# Autodesk Inventor assembly: chassis
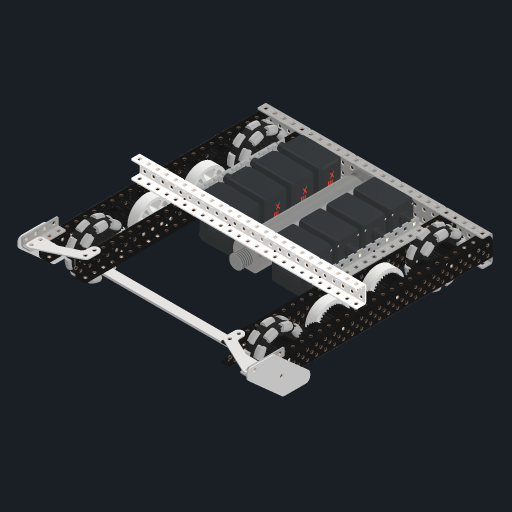
[picture p0: Inventor's stored thumbnail of the model, 512x512]
Saved by Autodesk Inventor 2024.2 (Build 282272000, 272)
## iProperties
Created: 2024-01-28
Part Number: chassis
Document SubType Name: Assembly
Designer: reima
Mass: 1228.84 g
Surface Area: 6404.9 cm^2
Volume: 505.466 cm^3
Density: 2.43111 g/cm^3
Author: reima
## Documents named in this file (15)
- O:\cad\61002g-cad\subasm\chassis.iam
- O:\cad\61002g-cad\VEX parts\Structure\C Channel\Aluminum 1x2x1\Alu C 1x2x1x25.ipt
- O:\cad\61002g-cad\VEX parts\Structure\C Channel\Aluminum 1x3x1\Alu C 1x3x1x25.ipt
- O:\cad\61002g-cad\subasm\omniAsemb.iam
- O:\cad\61002g-cad\subasm\flexMid.iam
- O:\cad\61002g-cad\VEX parts\Motion\Gears\LS 36T Gear.ipt
- O:\cad\61002g-cad\plastic parts\6inSleds.ipt
- O:\cad\61002g-cad\VEX parts\Structure\Angle\Aluminum 1x1\Alu Angle 1x1x4.ipt
- O:\cad\61002g-cad\plastic parts\frontgussets.ipt
- O:\cad\61002g-cad\VEX parts\Electronics\V5 Motor.ipt
- O:\cad\61002g-cad\plastic parts\undersideStrip.ipt
- O:\cad\61002g-cad\VEX parts\Structure\C Channel\Aluminum 1x2x1 Half\Alu Half C 1x2x1x10\Alu Half C 1x2x1x10.ipt
- O:\cad\61002g-cad\VEX parts\Structure\C Channel\Aluminum 1x2x1 Half\Alu Half C 1x2x1x10.ipt
- O:\cad\61002g-cad\VEX parts\Motion\Pneumatics\Reservoir.ipt
- O:\cad\61002g-cad\VEX parts\Miscellaneous\iw_metal_02.bmp
## Components (38 placed, 12 different names)
1. Alu C 1x2x1x25:1 — Insert:2, Mate:2, Insert:14, Insert:15, Insert:16, Insert:17, Mate:7, Mate:10, Flush:6, Flush:7, Insert:35
2. Alu C 1x2x1x25:2 — Insert:1, Mate:2, Insert:5, Insert:6, Insert:7, Insert:8, Insert:9, Insert:10, Insert:11, Insert:12, Angle:1, Insert:13, Mate:3, Mate:8
3. Alu C 1x3x1x25:1 — Insert:1, Insert:2, Angle:2, Flush:3, Insert:31
4. omniAsemb:3 [sub-assembly] — Insert:5
5. omniAsemb:6 [sub-assembly] — Insert:11
6. LS 36T Gear:4 — Insert:6
7. flexMid:5 [sub-assembly] — Insert:7
8. flexMid:6 [sub-assembly] — Insert:9
9. LS 36T Gear:5 — Insert:8
10. LS 36T Gear:6 — Insert:10
11. 6inSleds:2 — Insert:12, Angle:1
12. Alu Angle 1x1x4:1 — Insert:13, Mate:3
13. frontgussets:2 — Insert:14
14. V5 Motor:1 — Insert:15
15. V5 Motor:2 — Insert:16
16. V5 Motor:3 — Insert:17
17. Alu C 1x2x1x25:3 — Mate:5, Insert:27, Insert:28, Insert:29, Insert:30, Insert:33, Mate:9, Flush:4, Flush:5, Insert:36
18. Alu C 1x2x1x25:4 — Mate:5, Insert:18, Insert:19, Insert:20, Insert:21, Insert:22, Insert:23, Insert:24, Insert:25, Angle:3, Mate:6, Insert:26, Insert:31, Insert:34
19. omniAsemb:7 [sub-assembly] — Insert:18
20. omniAsemb:8 [sub-assembly] — Insert:19
21. LS 36T Gear:7 — Insert:20
22. flexMid:7 [sub-assembly] — Insert:21
23. flexMid:8 [sub-assembly] — Insert:22
24. LS 36T Gear:8 — Insert:23
25. LS 36T Gear:9 — Insert:24
26. 6inSleds:3 — Insert:25, Angle:3
27. Alu Angle 1x1x4:2 — Mate:6, Insert:26, Insert:32
28. frontgussets:3 — Insert:27, Insert:32
29. V5 Motor:4 — Insert:28
30. V5 Motor:5 — Insert:29
31. V5 Motor:6 — Insert:30
32. undersideStrip:2 — Insert:33, Mate:7
33. Alu C 1x2x1x25:5 — Insert:34, Mate:8, Mate:11, Mate:12
34. Alu Half C 1x2x1x10:1 — Mate:10, Flush:6, Flush:7
35. Alu Half C 1x2x1x10:2 — Mate:9, Flush:4, Flush:5
36. V5 Motor:7 — Insert:35
37. V5 Motor:8 — Insert:36
38. Reservoir:1 — Mate:11, Mate:12
## Relationships (52: Insert 34, Mate 10, Flush 5, Angle 3)
- Insert:1 (3.175 mm): Alu C 1x2x1x25:2 ↔ Alu C 1x3x1x25:1
- Insert:2 (3.175 mm): Alu C 1x2x1x25:1 ↔ Alu C 1x3x1x25:1
- Mate:2: Alu C 1x2x1x25:1 ↔ Alu C 1x2x1x25:2
- Insert:5 (13.4938 mm): Alu C 1x2x1x25:2 ↔ omniAsemb:3
- Insert:6 (13.4938 mm): Alu C 1x2x1x25:2 ↔ LS 36T Gear:4
- Insert:7 (13.4938 mm): Alu C 1x2x1x25:2 ↔ flexMid:5
- Insert:8 (13.4938 mm): Alu C 1x2x1x25:2 ↔ LS 36T Gear:5
- Insert:9 (13.4938 mm): Alu C 1x2x1x25:2 ↔ flexMid:6
- Insert:10 (13.4938 mm): Alu C 1x2x1x25:2 ↔ LS 36T Gear:6
- Insert:11 (13.4938 mm): Alu C 1x2x1x25:2 ↔ omniAsemb:6
- Insert:12: Alu C 1x2x1x25:2 ↔ 6inSleds:2
- Angle:1 (180 deg): Alu C 1x2x1x25:2 ↔ 6inSleds:2
- Insert:13: Alu C 1x2x1x25:2 ↔ Alu Angle 1x1x4:1
- Mate:3: Alu C 1x2x1x25:2 ↔ Alu Angle 1x1x4:1
- Insert:14 (1.5875 mm): Alu C 1x2x1x25:1 ↔ frontgussets:2
- Insert:15 (14.2875 mm): Alu C 1x2x1x25:1 ↔ V5 Motor:1
- Insert:16 (14.2875 mm): Alu C 1x2x1x25:1 ↔ V5 Motor:2
- Insert:17 (14.2875 mm): Alu C 1x2x1x25:1 ↔ V5 Motor:3
- Angle:2 (0 deg): Alu C 1x3x1x25:1
- Flush:3 (158.75 mm): Alu C 1x3x1x25:1
- Mate:5: Alu C 1x2x1x25:3 ↔ Alu C 1x2x1x25:4
- Insert:18 (13.4938 mm): Alu C 1x2x1x25:4 ↔ omniAsemb:7
- Insert:19 (13.4938 mm): Alu C 1x2x1x25:4 ↔ omniAsemb:8
- Insert:20 (13.4938 mm): Alu C 1x2x1x25:4 ↔ LS 36T Gear:7
- Insert:21 (13.4938 mm): Alu C 1x2x1x25:4 ↔ flexMid:7
- Insert:22 (13.4938 mm): Alu C 1x2x1x25:4 ↔ flexMid:8
- Insert:23 (13.4938 mm): Alu C 1x2x1x25:4 ↔ LS 36T Gear:8
- Insert:24 (13.4938 mm): Alu C 1x2x1x25:4 ↔ LS 36T Gear:9
- Insert:25: Alu C 1x2x1x25:4 ↔ 6inSleds:3
- Angle:3 (180 deg): Alu C 1x2x1x25:4 ↔ 6inSleds:3
- Mate:6: Alu C 1x2x1x25:4 ↔ Alu Angle 1x1x4:2
- Insert:26: Alu C 1x2x1x25:4 ↔ Alu Angle 1x1x4:2
- Insert:27 (1.5875 mm): Alu C 1x2x1x25:3 ↔ frontgussets:3
- Insert:28 (14.2875 mm): Alu C 1x2x1x25:3 ↔ V5 Motor:4
- Insert:29 (14.2875 mm): Alu C 1x2x1x25:3 ↔ V5 Motor:5
- Insert:30 (14.2875 mm): Alu C 1x2x1x25:3 ↔ V5 Motor:6
- Insert:31 (3.175 mm): Alu C 1x3x1x25:1 ↔ Alu C 1x2x1x25:4
- Insert:32: Alu Angle 1x1x4:2 ↔ frontgussets:3
- Insert:33: Alu C 1x2x1x25:3 ↔ undersideStrip:2
- Mate:7: Alu C 1x2x1x25:1 ↔ undersideStrip:2
- Insert:34 (6.35 mm): Alu C 1x2x1x25:4 ↔ Alu C 1x2x1x25:5
- Mate:8: Alu C 1x2x1x25:2 ↔ Alu C 1x2x1x25:5
- Mate:9: Alu C 1x2x1x25:3 ↔ Alu Half C 1x2x1x10:2
- Flush:4: Alu C 1x2x1x25:3 ↔ Alu Half C 1x2x1x10:2
- Flush:5: Alu C 1x2x1x25:3 ↔ Alu Half C 1x2x1x10:2
- Mate:10: Alu C 1x2x1x25:1 ↔ Alu Half C 1x2x1x10:1
- Flush:6: Alu C 1x2x1x25:1 ↔ Alu Half C 1x2x1x10:1
- Flush:7: Alu C 1x2x1x25:1 ↔ Alu Half C 1x2x1x10:1
- Insert:35 (14.2875 mm): Alu C 1x2x1x25:1 ↔ V5 Motor:7
- Insert:36 (14.2875 mm): Alu C 1x2x1x25:3 ↔ V5 Motor:8
- Mate:11: Alu C 1x2x1x25:5 ↔ Reservoir:1
- Mate:12: Alu C 1x2x1x25:5 ↔ Reservoir:1
